# Autodesk Inventor assembly: gripper full assembly
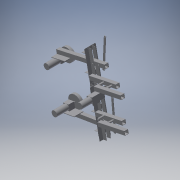
[picture p0: Inventor's stored thumbnail of the model, 180x180]
Saved by Autodesk Inventor 2016 SP2 (Build 200236200, 236)
## iProperties
Created: 2018-02-13
Part Number: gripper full assembly
Document SubType Name: Assembly
Designer: CAD
Author: CAD
## Documents named in this file (14)
- C:\Users\CAD\Documents\GitHub\FIRST-ROBOTICS-2018-5436-CAD\Robot\gripper\gripper full assembly.iam
- C:\Users\CAD\Documents\GitHub\FIRST-ROBOTICS-2018-5436-CAD\Robot\gripper\gripper main bracket.ipt
- C:\Users\CAD\Documents\GitHub\FIRST-ROBOTICS-2018-5436-CAD\Robot\gripper\gripper main arm.ipt
- C:\Users\CAD\Documents\GitHub\FIRST-ROBOTICS-2018-5436-CAD\Robot\gripper\gripper arm bracket.ipt
- C:\Users\CAD\Documents\GitHub\FIRST-ROBOTICS-2018-5436-CAD\Robot\gripper\gripper long spacers.ipt
- C:\Users\CAD\Documents\GitHub\FIRST-ROBOTICS-2018-5436-CAD\Robot\gripper\articulation motor mount spacer.ipt
- C:\Users\CAD\Documents\GitHub\FIRST-ROBOTICS-2018-5436-CAD\Robot\gripper\articulation motor mount.ipt
- C:\Users\CAD\Documents\GitHub\FIRST-ROBOTICS-2018-5436-CAD\Robot\gripper\motor spacer bracket.ipt
- C:\Users\CAD\Documents\GitHub\FIRST-ROBOTICS-2018-5436-CAD\Robot\gripper\NeveRest motor.ipt
- C:\Users\CAD\Documents\GitHub\FIRST-ROBOTICS-2018-5436-CAD\Robot\gripper\grabber wheels.ipt
- C:\Users\CAD\Documents\GitHub\FIRST-ROBOTICS-2018-5436-CAD\Robot\gripper\articulation motor 300 to 1.ipt
- C:\Users\CAD\Documents\GitHub\FIRST-ROBOTICS-2018-5436-CAD\Robot\gripper\articulation hub.ipt
- C:\Users\CAD\Documents\GitHub\FIRST-ROBOTICS-2018-5436-CAD\Robot\gripper\gripper limiter brackets.ipt
- C:\Users\CAD\Documents\GitHub\FIRST-ROBOTICS-2018-5436-CAD\Robot\gripper\grabber articulation arms.ipt
## Components (28 placed, 13 different names)
1. gripper main bracket:1 — Mate:1, Mate:2, Mate:3, Mate:4, Mate:30, Mate:31, Mate:32, Mate:33
2. gripper main bracket:2 — Mate:5, Mate:6, Mate:7, Mate:8, Mate:9, Mate:10, Mate:11, Mate:18, Mate:19, Flush:3, Flush:16, Flush:17, Flush:18, Flush:19, Flush:20
3. gripper main arm:1 — Mate:1, Mate:4, Mate:6, Mate:22, Flush:6, Flush:9, Flush:11, Flush:13, Mate:37
4. gripper main arm:2 — Mate:2, Mate:3, Mate:5, Mate:7, Mate:21, Flush:7, Flush:8, Flush:10, Flush:12, Mate:36
5. gripper arm bracket:1 — Mate:8, Mate:10, Mate:12, Mate:13, Flush:1
6. gripper arm bracket:2 — Mate:9, Mate:11, Mate:14, Mate:15, Flush:2
7. gripper long spacers:1 — Mate:15, Mate:16
8. gripper long spacers:2 — Mate:14
9. gripper long spacers:3 — Mate:13
10. gripper long spacers:4 — Mate:12, Mate:17
11. gripper arm bracket:3 — Mate:16, Flush:2
12. gripper arm bracket:4 — Mate:17, Flush:1
13. articulation motor mount spacer:1 — Mate:18, Mate:19, Flush:3, Mate:20, Flush:4, Flush:5
14. articulation motor mount:1 — Mate:20, Flush:4, Flush:5, Mate:27, Flush:21
15. motor spacer bracket:1 — Mate:22, Flush:6, Flush:9, Mate:24
16. motor spacer bracket:2 — Mate:21, Flush:7, Flush:8, Mate:23
17. NeveRest motor:1 — Mate:23, Flush:10, Flush:12, Mate:25, Flush:15
18. NeveRest motor:2 — Mate:24, Flush:11, Flush:13, Mate:26, Flush:14
19. grabber wheels:1 — Mate:25, Flush:15
20. grabber wheels:2 — Mate:26, Flush:14
21. articulation motor 300 to 1:1 — Mate:27, Flush:16, Mate:28, Mate:29, Flush:21
22. articulation hub:1 — Mate:28, Mate:29, Mate:34, Mate:35
23. gripper limiter brackets:1 — Mate:33, Flush:19
24. gripper limiter brackets:2 — Mate:32, Flush:20
25. gripper limiter brackets:3 — Mate:31, Flush:17
26. gripper limiter brackets:4 — Mate:30, Flush:18
27. grabber articulation arms:1 — Mate:35, Mate:37
28. grabber articulation arms:2 — Mate:34, Mate:36
## Relationships (58: Mate 37, Flush 21)
- Mate:1: gripper main bracket:1 ↔ gripper main arm:1
- Mate:2: gripper main bracket:1 ↔ gripper main arm:2
- Mate:3: gripper main bracket:1 ↔ gripper main arm:2
- Mate:4: gripper main bracket:1 ↔ gripper main arm:1
- Mate:5: gripper main bracket:2 ↔ gripper main arm:2
- Mate:6: gripper main bracket:2 ↔ gripper main arm:1
- Mate:7: gripper main bracket:2 ↔ gripper main arm:2
- Mate:8: gripper main bracket:2 ↔ gripper arm bracket:1
- Mate:9: gripper main bracket:2 ↔ gripper arm bracket:2
- Mate:10: gripper main bracket:2 ↔ gripper arm bracket:1
- Mate:11: gripper main bracket:2 ↔ gripper arm bracket:2
- Mate:12: gripper arm bracket:1 ↔ gripper long spacers:4
- Mate:13: gripper arm bracket:1 ↔ gripper long spacers:3
- Mate:14: gripper arm bracket:2 ↔ gripper long spacers:2
- Mate:15: gripper arm bracket:2 ↔ gripper long spacers:1
- Mate:16: gripper long spacers:1 ↔ gripper arm bracket:3
- Mate:17: gripper long spacers:4 ↔ gripper arm bracket:4
- Flush:1: gripper arm bracket:1 ↔ gripper arm bracket:4
- Flush:2: gripper arm bracket:2 ↔ gripper arm bracket:3
- Mate:18: gripper main bracket:2 ↔ articulation motor mount spacer:1
- Mate:19: gripper main bracket:2 ↔ articulation motor mount spacer:1
- Flush:3 (-215.9 mm): gripper main bracket:2 ↔ articulation motor mount spacer:1
- Mate:20: articulation motor mount spacer:1 ↔ articulation motor mount:1
- Flush:4: articulation motor mount spacer:1 ↔ articulation motor mount:1
- Flush:5: articulation motor mount spacer:1 ↔ articulation motor mount:1
- Mate:21: gripper main arm:2 ↔ motor spacer bracket:2
- Mate:22: gripper main arm:1 ↔ motor spacer bracket:1
- Flush:6: gripper main arm:1 ↔ motor spacer bracket:1
- Flush:7: gripper main arm:2 ↔ motor spacer bracket:2
- Flush:8: gripper main arm:2 ↔ motor spacer bracket:2
- Flush:9: gripper main arm:1 ↔ motor spacer bracket:1
- Mate:23: motor spacer bracket:2 ↔ NeveRest motor:1
- Mate:24: motor spacer bracket:1 ↔ NeveRest motor:2
- Flush:10: gripper main arm:2 ↔ NeveRest motor:1
- Flush:11: gripper main arm:1 ↔ NeveRest motor:2
- Flush:12: gripper main arm:2 ↔ NeveRest motor:1
- Flush:13: gripper main arm:1 ↔ NeveRest motor:2
- Mate:25: NeveRest motor:1 ↔ grabber wheels:1
- Mate:26: NeveRest motor:2 ↔ grabber wheels:2
- Flush:14: NeveRest motor:2 ↔ grabber wheels:2
- Flush:15: NeveRest motor:1 ↔ grabber wheels:1
- Mate:27: articulation motor mount:1 ↔ articulation motor 300 to 1:1
- Flush:16: gripper main bracket:2 ↔ articulation motor 300 to 1:1
- Mate:28: articulation motor 300 to 1:1 ↔ articulation hub:1
- Mate:29: articulation motor 300 to 1:1 ↔ articulation hub:1
- Mate:30: gripper main bracket:1 ↔ gripper limiter brackets:4
- Mate:31: gripper main bracket:1 ↔ gripper limiter brackets:3
- Mate:32: gripper main bracket:1 ↔ gripper limiter brackets:2
- Mate:33: gripper main bracket:1 ↔ gripper limiter brackets:1
- Flush:17: gripper main bracket:2 ↔ gripper limiter brackets:3
- Flush:18: gripper main bracket:2 ↔ gripper limiter brackets:4
- Flush:19: gripper main bracket:2 ↔ gripper limiter brackets:1
- Flush:20: gripper main bracket:2 ↔ gripper limiter brackets:2
- Flush:21 (31.75 mm): articulation motor mount:1 ↔ articulation motor 300 to 1:1
- Mate:34: articulation hub:1 ↔ grabber articulation arms:2
- Mate:35: articulation hub:1 ↔ grabber articulation arms:1
- Mate:36: gripper main arm:2 ↔ grabber articulation arms:2
- Mate:37: gripper main arm:1 ↔ grabber articulation arms:1
